# Autodesk Inventor assembly: ForeArm_
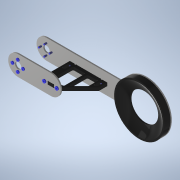
[picture p0: Inventor's stored thumbnail of the model, 180x180]
Saved by Autodesk Inventor 2020.4 (Build 244396000, 396)
## iProperties
Created: 2022-01-10
Part Number: ForeArm_
Document SubType Name: Assembly
Designer: Masato Kubotera
Author: Masato Kubotera
## Documents named in this file (9)
- C:\Users\Masato\Documents\Inventor\CIT Brains_Inventor\OpenPlatform_ver3_0 - ve4_1 branch\UpperBody\Arm\ForeArm_.iam
- C:\Users\Masato\Documents\Inventor\CIT Brains_Inventor\OpenPlatform_ver3_0 - ve4_1 branch\UpperBody\Arm\ForeArm_outside_frame_.ipt
- C:\Users\Masato\Documents\Inventor\CIT Brains_Inventor\OpenPlatform_ver3_0 - ve4_1 branch\UpperBody\Arm\Hand_.ipt
- C:\Users\Masato\Documents\Inventor\CIT Brains_Inventor\OpenPlatform_ver3_0 - ve4_1 branch\UpperBody\Arm\ForeArm_inside_frame_.ipt
- C:\Users\Masato\Documents\Inventor\CIT Brains_Inventor\OpenPlatform_ver3_0 - ve4_1 branch\Ready_Made\InsertNut\UD-43040.ipt
- C:\Users\Masato\Documents\Inventor\CIT Brains_Inventor\OpenPlatform_ver3_0 - ve4_1 branch\Ready_Made\Screw\M3-6.ipt
- C:\Users\Masato\Documents\Inventor\CIT Brains_Inventor\OpenPlatform_ver3_0 - ve4_1 branch\Ready_Made\Screw\M2_6-6.ipt
- C:\Users\Masato\Documents\Inventor\CIT Brains_Inventor\OpenPlatform_ver3_0 - ve4_1 branch\Ready_Made\InsertNut\IRU-304SW.ipt
- C:\Users\Masato\Documents\Inventor\CIT Brains_Inventor\OpenPlatform_ver3_0 - ve4_1 branch\UpperBody\Arm\ForeArm_diagonal_.ipt
## Components (32 placed, 8 different names)
1. ForeArm_outside_frame_:1 — 挿入:7, 挿入:8, 挿入:9, 挿入:10, 挿入:11, 挿入:12, 挿入:13, 挿入:14, 挿入:15, 挿入:16, 挿入:17, 挿入:18, 挿入:23, 挿入:24, 挿入:27, 挿入:28, 挿入:31, 挿入:32, 挿入:33, 挿入:34, メイト:1, メイト:2, フラッシュ:1
2. Hand_:1 — 挿入:1, 挿入:2, 挿入:3, 挿入:4, 挿入:5, 挿入:6
3. ForeArm_inside_frame_:1 — 挿入:25, 挿入:26, 挿入:29, 挿入:30, 挿入:35, 挿入:36, 挿入:37, 挿入:38
4. UD-43040:1 — 挿入:1, 挿入:7
5. UD-43040:2 — 挿入:2, 挿入:8
6. UD-43040:3 — 挿入:3, 挿入:9
7. UD-43040:4 — 挿入:4, 挿入:10
8. UD-43040:5 — 挿入:5, 挿入:11
9. UD-43040:6 — 挿入:6, 挿入:12
10. M3-6:1 — 挿入:13
11. M3-6:2 — 挿入:14
12. M3-6:3 — 挿入:15
13. M3-6:4 — 挿入:16
14. M3-6:5 — 挿入:17
15. M3-6:6 — 挿入:18
16. M2_6-6:1 — 挿入:31
17. M2_6-6:2 — 挿入:32
18. M2_6-6:3 — 挿入:33
19. M2_6-6:4 — 挿入:34
20. M2_6-6:5 — 挿入:35
21. M2_6-6:6 — 挿入:36
22. M2_6-6:7 — 挿入:37
23. M2_6-6:8 — 挿入:38
24. M3-6:7 — 挿入:27
25. M3-6:8 — 挿入:28
26. M3-6:9 — 挿入:29
27. M3-6:10 — 挿入:30
28. IRU-304SW:1 — 挿入:19, 挿入:23
29. IRU-304SW:2 — 挿入:20, 挿入:24
30. IRU-304SW:3 — 挿入:21, 挿入:25
31. IRU-304SW:4 — 挿入:22, 挿入:26
32. ForeArm_diagonal_:1 — 挿入:19, 挿入:20, 挿入:21, 挿入:22
## Relationships (41: Insert 38, Mate 2, Flush 1)
- 挿入:1 [Insert]: Hand_:1 ↔ UD-43040:1
- 挿入:2 [Insert]: Hand_:1 ↔ UD-43040:2
- 挿入:3 [Insert]: Hand_:1 ↔ UD-43040:3
- 挿入:4 [Insert]: Hand_:1 ↔ UD-43040:4
- 挿入:5 [Insert]: Hand_:1 ↔ UD-43040:5
- 挿入:6 [Insert]: Hand_:1 ↔ UD-43040:6
- 挿入:7 [Insert]: ForeArm_outside_frame_:1 ↔ UD-43040:1
- 挿入:8 [Insert]: ForeArm_outside_frame_:1 ↔ UD-43040:2
- 挿入:9 [Insert]: ForeArm_outside_frame_:1 ↔ UD-43040:3
- 挿入:10 [Insert]: ForeArm_outside_frame_:1 ↔ UD-43040:4
- 挿入:11 [Insert]: ForeArm_outside_frame_:1 ↔ UD-43040:5
- 挿入:12 [Insert]: ForeArm_outside_frame_:1 ↔ UD-43040:6
- 挿入:13 [Insert]: ForeArm_outside_frame_:1 ↔ M3-6:1
- 挿入:14 [Insert]: ForeArm_outside_frame_:1 ↔ M3-6:2
- 挿入:15 [Insert]: ForeArm_outside_frame_:1 ↔ M3-6:3
- 挿入:16 [Insert]: ForeArm_outside_frame_:1 ↔ M3-6:4
- 挿入:17 [Insert]: ForeArm_outside_frame_:1 ↔ M3-6:5
- 挿入:18 [Insert]: ForeArm_outside_frame_:1 ↔ M3-6:6
- 挿入:19 [Insert]: IRU-304SW:1 ↔ ForeArm_diagonal_:1
- 挿入:20 [Insert]: IRU-304SW:2 ↔ ForeArm_diagonal_:1
- 挿入:21 [Insert]: IRU-304SW:3 ↔ ForeArm_diagonal_:1
- 挿入:22 [Insert]: IRU-304SW:4 ↔ ForeArm_diagonal_:1
- 挿入:23 [Insert]: ForeArm_outside_frame_:1 ↔ IRU-304SW:1
- 挿入:24 [Insert]: ForeArm_outside_frame_:1 ↔ IRU-304SW:2
- 挿入:25 [Insert]: ForeArm_inside_frame_:1 ↔ IRU-304SW:3
- 挿入:26 [Insert]: ForeArm_inside_frame_:1 ↔ IRU-304SW:4
- 挿入:27 [Insert]: ForeArm_outside_frame_:1 ↔ M3-6:7
- 挿入:28 [Insert]: ForeArm_outside_frame_:1 ↔ M3-6:8
- 挿入:29 [Insert]: ForeArm_inside_frame_:1 ↔ M3-6:9
- 挿入:30 [Insert]: ForeArm_inside_frame_:1 ↔ M3-6:10
- 挿入:31 [Insert]: ForeArm_outside_frame_:1 ↔ M2_6-6:1
- 挿入:32 [Insert]: ForeArm_outside_frame_:1 ↔ M2_6-6:2
- 挿入:33 [Insert]: ForeArm_outside_frame_:1 ↔ M2_6-6:3
- 挿入:34 [Insert]: ForeArm_outside_frame_:1 ↔ M2_6-6:4
- 挿入:35 [Insert]: ForeArm_inside_frame_:1 ↔ M2_6-6:5
- 挿入:36 [Insert]: ForeArm_inside_frame_:1 ↔ M2_6-6:6
- 挿入:37 [Insert]: ForeArm_inside_frame_:1 ↔ M2_6-6:7
- 挿入:38 [Insert]: ForeArm_inside_frame_:1 ↔ M2_6-6:8
- メイト:1 [Mate]: ForeArm_outside_frame_:1
- メイト:2 [Mate]: ForeArm_outside_frame_:1
- フラッシュ:1 [Flush]: ForeArm_outside_frame_:1
